# Autodesk Inventor assembly: Assembly Rotation mechanism
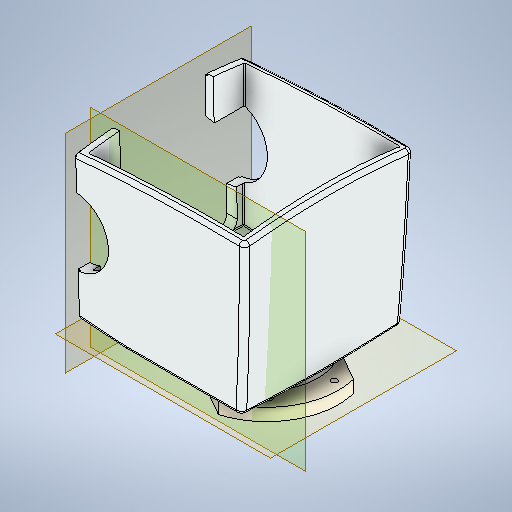
[picture p0: Inventor's stored thumbnail of the model, 512x512]
Saved by Autodesk Inventor 2025 (Build 290162000, 162)
## iProperties
Created: 2025-01-03
Part Number: Assembly Rotation mechanism
Document SubType Name: Assembly
Designer: marco.benkert
Author: marco.benkert
## Documents named in this file (6)
- O:\Inventor SanaBike Series\SanaBike 500&1000 Modifield\Rotation Mechanism\Assembly Rotation mechanism.iam
- O:\Inventor SanaBike Series\SanaBike 500&1000 Modifield\Rotation Mechanism\27-30-400 Bearing, Housing Measuring Head.ipt
- O:\Inventor SanaBike Series\SanaBike 500&1000 Modifield\Rotation Mechanism\35-30-xxx Plain Bearing Socket.ipt
- O:\Inventor SanaBike Series\SanaBike 500&1000 Modifield\Rotation Mechanism\25-30-100  Handlebar Cover.ipt
- O:\Inventor SanaBike Series\SanaBike 500&1000 Modifield\Rotation Mechanism\Passscheibe 40x50x1,2 - DIN 988 (ArtNr. 42-03-007)\Passscheibe 40x50x1,2 - DIN 988 (ArtNr. 42-03-007).ipt
- O:\Inventor SanaBike Series\SanaBike 500&1000 Modifield\Rotation Mechanism\Linsenflanschkopf (ecosyn-fix) M4x8 BN4825 (40-08-015)\Linsenflanschkopf (ecosyn-fix) M4x8 BN4825 (40-08-015).ipt
## Components (8 placed, 5 different names)
1. 27-30-400 Bearing, Housing Measuring Head:1 — Passend:6, Fluchtend:1, Passend:7, Passend:10, Fluchtend:2
2. 35-30-xxx Plain Bearing Socket:1 — Drehbar:1, Passend:6, Fluchtend:1
3. 25-30-100  Handlebar Cover:1 — Drehbar:1, Passend:8, Passend:9, Passend:11, Passend:12, Passend:14, Passend:16
4. Passscheibe 40x50x1,2 - DIN 988 (ArtNr. 42-03-007):1 — Passend:7, Passend:8, Passend:13, Passend:15, Passend:17
5. Linsenflanschkopf (ecosyn-fix) M4x8 BN4825 (40-08-015):1 — Passend:12, Passend:13
6. Linsenflanschkopf (ecosyn-fix) M4x8 BN4825 (40-08-015):2 — Passend:16, Passend:17
7. Linsenflanschkopf (ecosyn-fix) M4x8 BN4825 (40-08-015):3 — Passend:14, Passend:15
8. Passscheibe 40x50x1,2 - DIN 988 (ArtNr. 42-03-007):2 — Passend:9, Passend:10
## Relationships (15: Mate 12, Flush 2, RevoluteJoint 1)
- Drehbar:1 [RevoluteJoint]: 35-30-xxx Plain Bearing Socket:1 ↔ 25-30-100  Handlebar Cover:1
- Passend:6 [Mate]: 27-30-400 Bearing, Housing Measuring Head:1 ↔ 35-30-xxx Plain Bearing Socket:1
- Fluchtend:1 [Flush]: 27-30-400 Bearing, Housing Measuring Head:1 ↔ 35-30-xxx Plain Bearing Socket:1
- Passend:7 [Mate]: 27-30-400 Bearing, Housing Measuring Head:1 ↔ Passscheibe 40x50x1,2 - DIN 988 (ArtNr. 42-03-007):1
- Passend:8 [Mate]: 25-30-100  Handlebar Cover:1 ↔ Passscheibe 40x50x1,2 - DIN 988 (ArtNr. 42-03-007):1
- Passend:9 [Mate]: 25-30-100  Handlebar Cover:1 ↔ Passscheibe 40x50x1,2 - DIN 988 (ArtNr. 42-03-007):2
- Passend:10 [Mate]: 27-30-400 Bearing, Housing Measuring Head:1 ↔ Passscheibe 40x50x1,2 - DIN 988 (ArtNr. 42-03-007):2
- Fluchtend:2 [Flush]: 27-30-400 Bearing, Housing Measuring Head:1
- Passend:11 [Mate]: 25-30-100  Handlebar Cover:1
- Passend:12 [Mate]: 25-30-100  Handlebar Cover:1 ↔ Linsenflanschkopf (ecosyn-fix) M4x8 BN4825 (40-08-015):1
- Passend:13 [Mate]: Passscheibe 40x50x1,2 - DIN 988 (ArtNr. 42-03-007):1 ↔ Linsenflanschkopf (ecosyn-fix) M4x8 BN4825 (40-08-015):1
- Passend:14 [Mate]: 25-30-100  Handlebar Cover:1 ↔ Linsenflanschkopf (ecosyn-fix) M4x8 BN4825 (40-08-015):3
- Passend:15 [Mate]: Passscheibe 40x50x1,2 - DIN 988 (ArtNr. 42-03-007):1 ↔ Linsenflanschkopf (ecosyn-fix) M4x8 BN4825 (40-08-015):3
- Passend:16 [Mate]: 25-30-100  Handlebar Cover:1 ↔ Linsenflanschkopf (ecosyn-fix) M4x8 BN4825 (40-08-015):2
- Passend:17 [Mate]: Passscheibe 40x50x1,2 - DIN 988 (ArtNr. 42-03-007):1 ↔ Linsenflanschkopf (ecosyn-fix) M4x8 BN4825 (40-08-015):2
